# Autodesk Inventor assembly: PillowAssembly
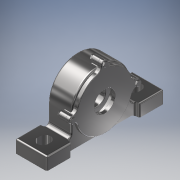
[picture p0: Inventor's stored thumbnail of the model, 180x180]
Saved by Autodesk Inventor 2018 (Build 220112000, 112)
## iProperties
Created: 2017-10-18
Part Number: PillowAssembly
Document SubType Name: Assembly
Designer: Bryce Richards
Mass: 1130.22 g
Surface Area: 490.469 cm^2
Volume: 143.977 cm^3
Density: 7.85 g/cm^3
Author: Bryce Richards
## Documents named in this file (6)
- C:\Users\P136265\Documents\mecanum-cad\PillowAssembly.iam
- C:\Users\P136265\Documents\mecanum-cad\MecanumPillowBlock.ipt
- C:\Users\P136265\Documents\mecanum-cad\PillowCover.ipt
- C:\Users\P136265\Documents\mecanum-cad\Inventor\Content Center Files\R2018\en-US\AS 1110\AS 1110 - M3 x 16.ipt
- C:\Users\P136265\Documents\mecanum-cad\Inventor\Content Center Files\R2018\en-US\AS 1474(1)\AS 1474 - M3.5(1).ipt
- C:\Users\P136265\Documents\Inventor\Content Center Files\R2018\en-US\DIN 625 SKF(4)\DIN 625 SKF - SKF E2.6304-2Z.ipt
## Components (9 placed, 5 different names)
1. MecanumPillowBlock:1 — Insert:1, Insert:5, Insert:6, Insert:7
2. DIN 625 SKF- with two Z shields SKF E2.6304-2Z:1 — Insert:1
3. PillowCover:1 — Insert:2, Insert:3, Insert:4
4. AS 1110 - Metric M3 x 16:1 — Insert:2
5. AS 1110 - Metric M3 x 16:2 — Insert:3
6. AS 1110 - Metric M3 x 16:3 — Insert:4
7. AS 1474 - Metric M3.5:1 — Insert:5
8. AS 1474 - Metric M3.5:2 — Insert:6
9. AS 1474 - Metric M3.5:3 — Insert:7
## Relationships (7: Insert 7)
- Insert:1: MecanumPillowBlock:1 ↔ DIN 625 SKF- with two Z shields SKF E2.6304-2Z:1
- Insert:2: PillowCover:1 ↔ AS 1110 - Metric M3 x 16:1
- Insert:3: PillowCover:1 ↔ AS 1110 - Metric M3 x 16:2
- Insert:4: PillowCover:1 ↔ AS 1110 - Metric M3 x 16:3
- Insert:5: MecanumPillowBlock:1 ↔ AS 1474 - Metric M3.5:1
- Insert:6: MecanumPillowBlock:1 ↔ AS 1474 - Metric M3.5:2
- Insert:7: MecanumPillowBlock:1 ↔ AS 1474 - Metric M3.5:3
